# Autodesk Inventor assembly: ProbeHead V5 - Assembly
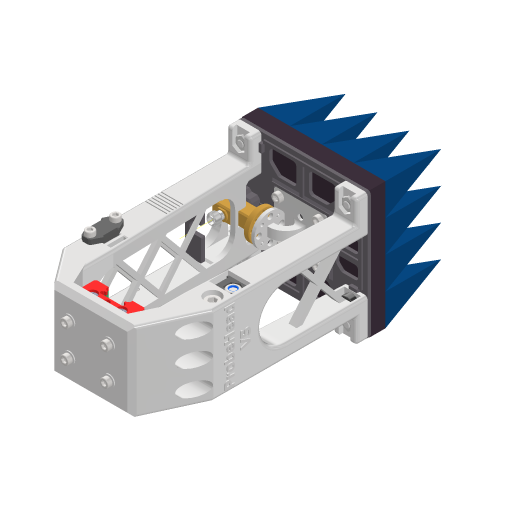
[picture p0: Inventor's stored thumbnail of the model, 512x512]
Saved by Autodesk Inventor 2023.2 (Build 272271000, 271)
## iProperties
Created: 2024-02-09
Part Number: ProbeHead V5 - Assembly
Document SubType Name: Assembly
Designer: Nils Bade
Author: Nils Bade
## Documents named in this file (21)
- C:\Users\nilsb\Documents\Inventor\Projektarbeit-Bade\RatRig_modified\ProbeHead\ProbeHead V5 - Assembly.iam
- C:\Users\nilsb\Documents\Inventor\Projektarbeit-Bade\RatRig_modified\MGN15 Linear-Rail-Block.ipt
- C:\Users\nilsb\Documents\Inventor\Projektarbeit-Bade\RatRig_Standards\face_belt_grabber v2.ipt
- C:\Users\nilsb\Documents\Inventor\Projektarbeit-Bade\Schrauben\Cap Head Screw M3x12 v2.ipt
- C:\Users\nilsb\Documents\Inventor\Projektarbeit-Bade\RatRig_Standards\Hex Nut - M3 v2.ipt
- C:\Users\nilsb\Documents\Inventor\Projektarbeit-Bade\Schrauben\Cap Head Screw M5x40 v2.ipt
- C:\Users\nilsb\Documents\Inventor\Projektarbeit-Bade\RatRig_Standards\Hex Locking Nut - M5 v2.ipt
- C:\Users\nilsb\Documents\Inventor\Projektarbeit-Bade\Schrauben\Washer Simple M3 - DIN6902.ipt
- C:\Users\nilsb\Documents\Inventor\Projektarbeit-Bade\RatRig_modified\ProbeHead\Wire2Probe_Eravant_SWC-15VF-R1-V.ipt
- C:\Users\nilsb\Documents\Inventor\Projektarbeit-Bade\RatRig_modified\core_xy_belt_grabber_Bade.ipt
- C:\Users\nilsb\Documents\Inventor\Projektarbeit-Bade\RatRig_modified\ProbeHead\ProbeHead_Kabelfixieung_V1.ipt
- C:\Users\nilsb\Documents\Inventor\Projektarbeit-Bade\Enclosure\Magnet-RatrigEnclosure.ipt
- C:\Users\nilsb\Documents\Inventor\Projektarbeit-Bade\RatRig_Standards\Hex Nut - M4 DIN934.ipt
- C:\Users\nilsb\Documents\Inventor\Projektarbeit-Bade\Schrauben\Cap Head Screw M4x8 - DIN912.ipt
- C:\Users\nilsb\Documents\Inventor\Projektarbeit-Bade\RatRig_modified\ProbeHead\ProbeHead-Arms V5.ipt
- C:\Users\nilsb\Documents\Inventor\Projektarbeit-Bade\RatRig_modified\ProbeHead\ProbeAntennas\ProbeAntenna_AdapterPlate_V1.ipt
- C:\Users\nilsb\Documents\Inventor\Projektarbeit-Bade\RatRig_modified\ProbeHead\ProbeAntennas\ProbeAntenna_AdapterRWG_V1_Assembled.iam
- C:\Users\nilsb\Documents\Inventor\Projektarbeit-Bade\RatRig_Standards\Cap Head Screw M3x8 v2.ipt
- C:\Users\nilsb\Documents\Inventor\Projektarbeit-Bade\RatRig_modified\ProbeHead\ProbeAntennas\IHFStandardParts\RWG-V_Band Backingplate.ipt
- C:\Users\nilsb\Documents\Inventor\Projektarbeit-Bade\RatRig_modified\ProbeHead\ProbeAntennas\ProbeAntenna_V3_Assembled.ipt
- C:\Users\nilsb\Documents\Inventor\Projektarbeit-Bade\Enclosure\Absorber\Absorber - ProbeHead_OERWGprobe.ipt
## Components (54 placed, 20 different names)
1. ProbeHead-Arms_V5:1 — Passend:102, Fluchtend:5, Passend:103, Passend:104, Passend:105, Passend:110, Passend:111, Passend:112, Winkel:17
2. core_xy_belt_grabber_Bade:2
3. core_xy_belt_grabber_Bade:1
4. MGN15 Linear-Rail-Block:1
5. face_belt_grabber v2:1 — Passend:16, Passend:17, Passend:18, Passend:19
6. face_belt_grabber v2:2 — Passend:12, Passend:13, Passend:14, Passend:15
7. Cap Head Screw M3x12 v2:1 — Passend:16, Passend:18, Passend:20
8. Cap Head Screw M3x12 v2:2 — Passend:17, Passend:19, Passend:21
9. Cap Head Screw M3x12 v2:3 — Passend:12, Passend:14, Passend:22
10. Cap Head Screw M3x12 v2:4 — Passend:13, Passend:15, Passend:23
11. Hex Nut - M3 v2:1 — Passend:20
12. Hex Nut - M3 v2:2 — Passend:23
13. Hex Nut - M3 v2:3 — Passend:22
14. Hex Nut - M3 v2:4 — Passend:21
15. Cap Head Screw M5x40 v2:1 — Passend:34
16. Cap Head Screw M5x40 v2:2
17. Hex Locking Nut - M5 v2:1
18. Hex Locking Nut - M5 v2:2 — Passend:34
19. Washer Simple M3 - DIN6902:1 — Passend:59
20. Washer Simple M3 - DIN6902:2 — Passend:56
21. Washer Simple M3 - DIN6902:3 — Passend:58
22. Washer Simple M3 - DIN6902:4 — Passend:57
23. Cap Head Screw M3x12 v2:5 — Passend:59
24. Cap Head Screw M3x12 v2:6 — Passend:58
25. Cap Head Screw M3x12 v2:7 — Passend:56
26. Cap Head Screw M3x12 v2:8 — Passend:57
27. Wire2Probe_Eravant_SWC-15VF-R1-V:1 — Fluchtend:6, Fluchtend:7, Passend:106
28. ProbeHead_Kabelfixieung_V1:1 — Passend:102, Fluchtend:5, Passend:103
29. Magnet-RatrigEnclosure:1
30. Magnet-RatrigEnclosure:2
31. Magnet-RatrigEnclosure:3
32. Magnet-RatrigEnclosure:4
33. Magnet-RatrigEnclosure:5
34. Hex Nut - M4 DIN934:1 — Passend:101, Passend:104
35. Hex Nut - M4 DIN934:2 — Passend:98
36. Hex Nut - M4 DIN934:3 — Passend:99, Passend:105
37. Hex Nut - M4 DIN934:4 — Passend:100
38. Cap Head Screw M4x8 - DIN912:1 — Passend:99, Passend:132
39. Cap Head Screw M4x8 - DIN912:2 — Passend:98, Passend:129
40. Cap Head Screw M4x8 - DIN912:3 — Passend:101, Passend:130
41. Cap Head Screw M4x8 - DIN912:4 — Passend:100, Passend:131
42. ProbeAntenna_AdapterPlate_V1:1 — Passend:107, Passend:108, Passend:109, Passend:110, Passend:111, Passend:112, Passend:121, Passend:122, Passend:123, Passend:124, Passend:129, Passend:130, Passend:131, Passend:132, Passend:140
43. ProbeAntenna_AdapterRWG_V1_Assembled:1 [sub-assembly] — Fluchtend:6, Fluchtend:7, Passend:106, Passend:107, Passend:108, Passend:109, Passend:113, Passend:114, Passend:115, Passend:116, Passend:117, Passend:118, Passend:119, Passend:120, Passend:133, Passend:134, Passend:135
44. Cap Head Screw M3x8 v2:1 — Passend:113, Passend:119, Passend:128
45. Cap Head Screw M3x8 v2:2 — Passend:114, Passend:118, Passend:127
46. Cap Head Screw M3x8 v2:3 — Passend:116, Passend:120, Passend:125
47. Cap Head Screw M3x8 v2:4 — Passend:115, Passend:117, Passend:126
48. Hex Nut - M3 v2:5 — Passend:122, Passend:127
49. Hex Nut - M3 v2:6 — Passend:121, Passend:126
50. Hex Nut - M3 v2:7 — Passend:123, Passend:128
51. Hex Nut - M3 v2:8 — Passend:124, Passend:125
52. RWG-V_Band Backingplate:1 — Passend:133, Passend:134, Passend:135
53. ProbeAntenna_V3_Assembled:1 — Passend:139
54. Absorber - ProbeHead_OERWGprobe:1 — Winkel:17, Passend:139, Passend:140
## Relationships (128: Mate 110, Angle 13, Flush 5)
- [Mate]: ProbeHead-Arms_V5:1 ↔ MGN15 Linear-Rail-Block:1
- [Mate]: ProbeHead-Arms_V5:1 ↔ MGN15 Linear-Rail-Block:1
- [Mate]: ProbeHead-Arms_V5:1 ↔ MGN15 Linear-Rail-Block:1
- [Mate]: ProbeHead-Arms_V5:1 ↔ core_xy_belt_grabber_Bade:1
- [Angle] (0 deg): ProbeHead-Arms_V5:1 ↔ core_xy_belt_grabber_Bade:2
- [Mate]: ProbeHead-Arms_V5:1 ↔ core_xy_belt_grabber_Bade:2
- [Flush] (2 mm): ProbeHead-Arms_V5:1 ↔ core_xy_belt_grabber_Bade:2
- [Flush] (2 mm): ProbeHead-Arms_V5:1 ↔ core_xy_belt_grabber_Bade:1
- [Mate]: ProbeHead-Arms_V5:1 ↔ face_belt_grabber v2:2
- [Mate]: ProbeHead-Arms_V5:1 ↔ face_belt_grabber v2:2
- [Mate]: ProbeHead-Arms_V5:1 ↔ face_belt_grabber v2:1
- [Mate]: ProbeHead-Arms_V5:1 ↔ face_belt_grabber v2:1
- Passend:12 [Mate]: face_belt_grabber v2:2 ↔ Cap Head Screw M3x12 v2:3
- Passend:13 [Mate]: face_belt_grabber v2:2 ↔ Cap Head Screw M3x12 v2:4
- Passend:14 [Mate]: face_belt_grabber v2:2 ↔ Cap Head Screw M3x12 v2:3
- Passend:15 [Mate]: face_belt_grabber v2:2 ↔ Cap Head Screw M3x12 v2:4
- Passend:16 [Mate]: face_belt_grabber v2:1 ↔ Cap Head Screw M3x12 v2:1
- Passend:17 [Mate]: face_belt_grabber v2:1 ↔ Cap Head Screw M3x12 v2:2
- Passend:18 [Mate]: face_belt_grabber v2:1 ↔ Cap Head Screw M3x12 v2:1
- Passend:19 [Mate]: face_belt_grabber v2:1 ↔ Cap Head Screw M3x12 v2:2
- Passend:20 [Mate]: Cap Head Screw M3x12 v2:1 ↔ Hex Nut - M3 v2:1
- Passend:21 [Mate]: Cap Head Screw M3x12 v2:2 ↔ Hex Nut - M3 v2:4
- Passend:22 [Mate]: Cap Head Screw M3x12 v2:3 ↔ Hex Nut - M3 v2:3
- Passend:23 [Mate]: Cap Head Screw M3x12 v2:4 ↔ Hex Nut - M3 v2:2
- [Angle] (0 deg): ProbeHead-Arms_V5:1 ↔ Hex Nut - M3 v2:1
- [Angle] (0 deg): ProbeHead-Arms_V5:1 ↔ Hex Nut - M3 v2:3
- [Mate]: ProbeHead-Arms_V5:1 ↔ Hex Nut - M3 v2:3
- [Mate]: ProbeHead-Arms_V5:1 ↔ Hex Nut - M3 v2:2
- [Mate]: ProbeHead-Arms_V5:1 ↔ Hex Nut - M3 v2:1
- [Mate]: ProbeHead-Arms_V5:1 ↔ Hex Nut - M3 v2:4
- [Mate]: ProbeHead-Arms_V5:1 ↔ Cap Head Screw M5x40 v2:2
- [Mate]: ProbeHead-Arms_V5:1 ↔ Cap Head Screw M5x40 v2:1
- [Mate]: ProbeHead-Arms_V5:1 ↔ Cap Head Screw M5x40 v2:1
- [Mate]: ProbeHead-Arms_V5:1 ↔ Cap Head Screw M5x40 v2:2
- [Mate]: core_xy_belt_grabber_Bade:1 ↔ Hex Locking Nut - M5 v2:1
- [Mate]: core_xy_belt_grabber_Bade:1 ↔ Hex Locking Nut - M5 v2:1
- Passend:34 [Mate]: Cap Head Screw M5x40 v2:1 ↔ Hex Locking Nut - M5 v2:2
- [Angle] (0 deg): core_xy_belt_grabber_Bade:2 ↔ Hex Locking Nut - M5 v2:2
- [Mate]: core_xy_belt_grabber_Bade:2 ↔ Hex Locking Nut - M5 v2:2
- [Angle] (0 deg): core_xy_belt_grabber_Bade:1 ↔ Hex Locking Nut - M5 v2:1
- [Mate]: ProbeHead-Arms_V5:1 ↔ Washer Simple M3 - DIN6902:1
- [Mate]: ProbeHead-Arms_V5:1 ↔ Washer Simple M3 - DIN6902:2
- [Mate]: ProbeHead-Arms_V5:1 ↔ Washer Simple M3 - DIN6902:3
- [Mate]: ProbeHead-Arms_V5:1 ↔ Washer Simple M3 - DIN6902:4
- [Mate]: ProbeHead-Arms_V5:1 ↔ Washer Simple M3 - DIN6902:4
- [Mate]: ProbeHead-Arms_V5:1 ↔ Washer Simple M3 - DIN6902:2
- [Mate]: ProbeHead-Arms_V5:1 ↔ Washer Simple M3 - DIN6902:1
- [Mate]: ProbeHead-Arms_V5:1 ↔ Washer Simple M3 - DIN6902:3
- [Mate]: ProbeHead-Arms_V5:1 ↔ Cap Head Screw M3x12 v2:5
- [Mate]: ProbeHead-Arms_V5:1 ↔ Cap Head Screw M3x12 v2:6
- [Mate]: ProbeHead-Arms_V5:1 ↔ Cap Head Screw M3x12 v2:7
- [Mate]: ProbeHead-Arms_V5:1 ↔ Cap Head Screw M3x12 v2:8
- Passend:56 [Mate]: Washer Simple M3 - DIN6902:2 ↔ Cap Head Screw M3x12 v2:7
- Passend:57 [Mate]: Washer Simple M3 - DIN6902:4 ↔ Cap Head Screw M3x12 v2:8
- Passend:58 [Mate]: Washer Simple M3 - DIN6902:3 ↔ Cap Head Screw M3x12 v2:6
- Passend:59 [Mate]: Washer Simple M3 - DIN6902:1 ↔ Cap Head Screw M3x12 v2:5
- [Mate]: ProbeHead-Arms_V5:1 ↔ Cap Head Screw M3x12 v2:4
- [Mate]: ProbeHead-Arms_V5:1 ↔ Cap Head Screw M3x12 v2:2
- [Angle] (0 deg): ProbeHead-Arms_V5:1 ↔ Hex Nut - M3 v2:2
- [Angle] (0 deg): ProbeHead-Arms_V5:1 ↔ Hex Nut - M3 v2:4
- [Angle] (180 deg): ProbeHead-Arms_V5:1 ↔ core_xy_belt_grabber_Bade:1
- [Mate]: ProbeHead-Arms_V5:1 ↔ Magnet-RatrigEnclosure:1
- [Mate]: ProbeHead-Arms_V5:1 ↔ Magnet-RatrigEnclosure:4
- [Mate]: ProbeHead-Arms_V5:1 ↔ Magnet-RatrigEnclosure:3
- [Mate]: ProbeHead-Arms_V5:1 ↔ Magnet-RatrigEnclosure:2
- [Mate]: ProbeHead-Arms_V5:1 ↔ Magnet-RatrigEnclosure:4
- [Mate]: ProbeHead-Arms_V5:1 ↔ Magnet-RatrigEnclosure:1
- [Mate]: ProbeHead-Arms_V5:1 ↔ Magnet-RatrigEnclosure:2
- [Mate]: ProbeHead-Arms_V5:1 ↔ Magnet-RatrigEnclosure:3
- [Mate]: ProbeHead-Arms_V5:1 ↔ Magnet-RatrigEnclosure:5
- [Mate]: ProbeHead-Arms_V5:1 ↔ Magnet-RatrigEnclosure:5
- [Angle] (0 deg): ProbeHead-Arms_V5:1 ↔ Hex Nut - M4 DIN934:1
- [Angle] (0 deg): ProbeHead-Arms_V5:1 ↔ Hex Nut - M4 DIN934:2
- [Angle] (0 deg): ProbeHead-Arms_V5:1 ↔ Hex Nut - M4 DIN934:3
- [Angle] (0 deg): ProbeHead-Arms_V5:1 ↔ Hex Nut - M4 DIN934:4
- [Mate]: ProbeHead-Arms_V5:1 ↔ Hex Nut - M4 DIN934:4
- [Mate]: ProbeHead-Arms_V5:1 ↔ Hex Nut - M4 DIN934:3
- [Mate]: ProbeHead-Arms_V5:1 ↔ Hex Nut - M4 DIN934:2
- [Mate]: ProbeHead-Arms_V5:1 ↔ Hex Nut - M4 DIN934:1
- [Mate]: ProbeHead-Arms_V5:1 ↔ Cap Head Screw M4x8 - DIN912:4
- [Mate]: ProbeHead-Arms_V5:1 ↔ Cap Head Screw M4x8 - DIN912:2
- Passend:98 [Mate]: Hex Nut - M4 DIN934:2 ↔ Cap Head Screw M4x8 - DIN912:2
- Passend:99 [Mate]: Hex Nut - M4 DIN934:3 ↔ Cap Head Screw M4x8 - DIN912:1
- Passend:100 [Mate]: Hex Nut - M4 DIN934:4 ↔ Cap Head Screw M4x8 - DIN912:4
- Passend:101 [Mate]: Hex Nut - M4 DIN934:1 ↔ Cap Head Screw M4x8 - DIN912:3
- Passend:102 [Mate]: ProbeHead-Arms_V5:1 ↔ ProbeHead_Kabelfixieung_V1:1
- Fluchtend:5 [Flush]: ProbeHead-Arms_V5:1 ↔ ProbeHead_Kabelfixieung_V1:1
- Passend:103 [Mate] (16 mm): ProbeHead-Arms_V5:1 ↔ ProbeHead_Kabelfixieung_V1:1
- Passend:104 [Mate]: ProbeHead-Arms_V5:1 ↔ Hex Nut - M4 DIN934:1
- Passend:105 [Mate]: ProbeHead-Arms_V5:1 ↔ Hex Nut - M4 DIN934:3
- Fluchtend:6 [Flush]: Wire2Probe_Eravant_SWC-15VF-R1-V:1 ↔ ProbeAntenna_AdapterRWG_V1_Assembled:1
- Fluchtend:7 [Flush]: Wire2Probe_Eravant_SWC-15VF-R1-V:1 ↔ ProbeAntenna_AdapterRWG_V1_Assembled:1
- Passend:106 [Mate]: Wire2Probe_Eravant_SWC-15VF-R1-V:1 ↔ ProbeAntenna_AdapterRWG_V1_Assembled:1
- Passend:107 [Mate]: ProbeAntenna_AdapterPlate_V1:1 ↔ ProbeAntenna_AdapterRWG_V1_Assembled:1
- Passend:108 [Mate]: ProbeAntenna_AdapterPlate_V1:1 ↔ ProbeAntenna_AdapterRWG_V1_Assembled:1
- Passend:109 [Mate]: ProbeAntenna_AdapterPlate_V1:1 ↔ ProbeAntenna_AdapterRWG_V1_Assembled:1
- Passend:110 [Mate]: ProbeHead-Arms_V5:1 ↔ ProbeAntenna_AdapterPlate_V1:1
- Passend:111 [Mate]: ProbeHead-Arms_V5:1 ↔ ProbeAntenna_AdapterPlate_V1:1
- Passend:112 [Mate]: ProbeHead-Arms_V5:1 ↔ ProbeAntenna_AdapterPlate_V1:1
- Passend:113 [Mate]: ProbeAntenna_AdapterRWG_V1_Assembled:1 ↔ Cap Head Screw M3x8 v2:1
- Passend:114 [Mate]: ProbeAntenna_AdapterRWG_V1_Assembled:1 ↔ Cap Head Screw M3x8 v2:2
- Passend:115 [Mate]: ProbeAntenna_AdapterRWG_V1_Assembled:1 ↔ Cap Head Screw M3x8 v2:4
- Passend:116 [Mate]: ProbeAntenna_AdapterRWG_V1_Assembled:1 ↔ Cap Head Screw M3x8 v2:3
- Passend:117 [Mate]: ProbeAntenna_AdapterRWG_V1_Assembled:1 ↔ Cap Head Screw M3x8 v2:4
- Passend:118 [Mate]: ProbeAntenna_AdapterRWG_V1_Assembled:1 ↔ Cap Head Screw M3x8 v2:2
- Passend:119 [Mate]: ProbeAntenna_AdapterRWG_V1_Assembled:1 ↔ Cap Head Screw M3x8 v2:1
- Passend:120 [Mate]: ProbeAntenna_AdapterRWG_V1_Assembled:1 ↔ Cap Head Screw M3x8 v2:3
- Passend:121 [Mate]: ProbeAntenna_AdapterPlate_V1:1 ↔ Hex Nut - M3 v2:6
- Passend:122 [Mate]: ProbeAntenna_AdapterPlate_V1:1 ↔ Hex Nut - M3 v2:5
- Passend:123 [Mate]: ProbeAntenna_AdapterPlate_V1:1 ↔ Hex Nut - M3 v2:7
- Passend:124 [Mate]: ProbeAntenna_AdapterPlate_V1:1 ↔ Hex Nut - M3 v2:8
- Passend:125 [Mate]: Cap Head Screw M3x8 v2:3 ↔ Hex Nut - M3 v2:8
- Passend:126 [Mate]: Cap Head Screw M3x8 v2:4 ↔ Hex Nut - M3 v2:6
- Passend:127 [Mate]: Cap Head Screw M3x8 v2:2 ↔ Hex Nut - M3 v2:5
- Passend:128 [Mate]: Cap Head Screw M3x8 v2:1 ↔ Hex Nut - M3 v2:7
- Passend:129 [Mate]: Cap Head Screw M4x8 - DIN912:2 ↔ ProbeAntenna_AdapterPlate_V1:1
- Passend:130 [Mate]: Cap Head Screw M4x8 - DIN912:3 ↔ ProbeAntenna_AdapterPlate_V1:1
- Passend:131 [Mate]: Cap Head Screw M4x8 - DIN912:4 ↔ ProbeAntenna_AdapterPlate_V1:1
- Passend:132 [Mate]: Cap Head Screw M4x8 - DIN912:1 ↔ ProbeAntenna_AdapterPlate_V1:1
- Passend:133 [Mate]: ProbeAntenna_AdapterRWG_V1_Assembled:1 ↔ RWG-V_Band Backingplate:1
- Passend:134 [Mate]: ProbeAntenna_AdapterRWG_V1_Assembled:1 ↔ RWG-V_Band Backingplate:1
- Passend:135 [Mate]: ProbeAntenna_AdapterRWG_V1_Assembled:1 ↔ RWG-V_Band Backingplate:1
- [Mate]: ProbeAntenna_AdapterRWG_V1_Assembled:1 ↔ ProbeAntenna_V3_Assembled:1
- [Mate]: ProbeAntenna_AdapterRWG_V1_Assembled:1 ↔ ProbeAntenna_V3_Assembled:1
- [Mate]: ProbeAntenna_AdapterRWG_V1_Assembled:1 ↔ ProbeAntenna_V3_Assembled:1
- Winkel:17 [Angle] (0 deg): ProbeHead-Arms_V5:1 ↔ Absorber - ProbeHead_OERWGprobe:1
- Passend:139 [Mate]: ProbeAntenna_V3_Assembled:1 ↔ Absorber - ProbeHead_OERWGprobe:1
- Passend:140 [Mate]: ProbeAntenna_AdapterPlate_V1:1 ↔ Absorber - ProbeHead_OERWGprobe:1
